# Autodesk Inventor assembly: Frame
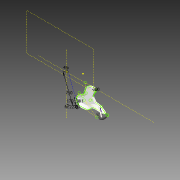
[picture p0: Inventor's stored thumbnail of the model, 180x180]
Saved by Autodesk Inventor 2016 (Build 200138000, 138)
## iProperties
Created: 2015-03-25
Part Number: Frame
Document SubType Name: Assembly
Designer: Yann
Author: Yann
## Documents named in this file (7)
- C:\Users\Yann\Documents\GitHub\Bikair_CAD\Source\Frame\Frame.iam
- C:\Users\Yann\Documents\GitHub\Bikair_CAD\Source\Frame\Frame_Generator.ipt
- C:\Users\Yann\Documents\GitHub\Bikair_CAD\Source\Frame\Pivots_Support.ipt
- C:\Users\Yann\Documents\GitHub\Bikair_CAD\Source\Frame\Rear_Strut_pivot_support.ipt
- C:\Users\Yann\Documents\GitHub\Bikair_CAD\Source\Front_Train\Headlight\Low_beam_optic.ipt
- C:\Users\Yann\Documents\GitHub\Bikair_CAD\Source\Frame\Saddle.ipt
- C:\Program Files (x86)\Common Files\Autodesk Shared\Materials\Textures\carbon-fiber--very-detailed.jpg
## Components (7 placed, 5 different names)
1. Frame_Generator:1 — Affleurement:2, Placage:1, Placage:2
2. Pivots_Support:1
3. Rear_Strut_pivot_support:1 — Flush:6, Flush:7, Flush:8
4. Low_beam_optic:1 — Mate:3
5. Low_beam_optic:2
6. Low_beam_optic:3
7. Saddle:2 — Flush:10
## Relationships (8: Flush 5, Mate 3)
- Affleurement:2 [Flush]: Frame_Generator:1
- Placage:1 [Mate]: Frame_Generator:1
- Placage:2 [Mate]: Frame_Generator:1
- Flush:6: Rear_Strut_pivot_support:1
- Flush:7: Rear_Strut_pivot_support:1
- Flush:8: Rear_Strut_pivot_support:1
- Mate:3: Low_beam_optic:1
- Flush:10: Saddle:2
